# Autodesk Inventor assembly: Tangent Plane
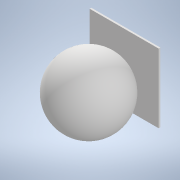
[picture p0: Inventor's stored thumbnail of the model, 180x180]
Saved by Autodesk Inventor 2020 (Build 240168000, 168)
## iProperties
Created: 2020-12-04
Part Number: Tangent Plane
Document SubType Name: Assembly
Designer: Ethan
Author: Ethan
## Documents named in this file (3)
- F:\Spring 2020 Honors Project\Tangent Plane.iam
- F:\Spring 2020 Honors Project\Plain.ipt
- F:\Spring 2020 Honors Project\Sphere.ipt
## Components (2 placed, 2 different names)
1. Plain:1 — Tangent:1
2. Sphere:1 — Tangent:1
## Relationships (1: Tangent 1)
- Tangent:1: Plain:1 ↔ Sphere:1
